# Autodesk Inventor assembly: ウィングユニット
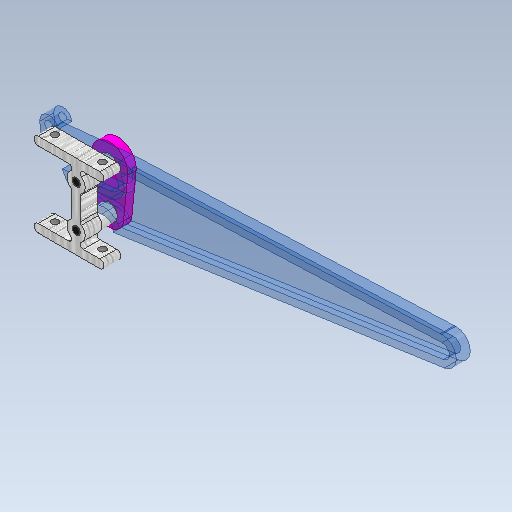
[picture p0: Inventor's stored thumbnail of the model, 512x512]
Saved by Autodesk Inventor 2020.2 (Build 242310000, 310)
## iProperties
Created: 2020-04-20
Part Number: ウィングユニット
Document SubType Name: Assembly
Designer: aoyama
Mass: 14.4308 g
Surface Area: 106.096 cm^2
Volume: 8.3252 cm^3
Density: 1.73339 g/cm^3
Author: aoyama
## Documents named in this file (6)
- C:\Users\aoyam\Desktop\SRDC_local\Inventor\二年機\Geminiβ\翼\WingUnitL.iam
- C:\Users\aoyam\Desktop\SRDC_local\Inventor\二年機\Geminiβ\翼\ウィング.ipt
- C:\Users\aoyam\Desktop\SRDC_local\Inventor\二年機\Geminiβ\翼\ウィング土台.ipt
- C:\Users\aoyam\Desktop\SRDC_local\Inventor\二年機\Geminiβ\翼\ウィング抑え.ipt
- C:\Users\aoyam\Desktop\SRDC_local\Inventor\二年機\Geminiβ\汎用部品\スペーサー中空M3L6アルミ.ipt
- C:\Users\aoyam\Desktop\SRDC_local\Inventor\二年機\Geminiβ\汎用部品\ネジボタンM3L15.ipt
## Components (7 placed, 5 different names)
1. ウィング:1 — 挿入:1
2. ウィング土台:1 — 挿入:1, 挿入:2, 挿入:3
3. ウィング抑え:1 — 挿入:4, 挿入:5, 挿入:6, 挿入:7
4. スペーサー中空M3L6アルミ:1 — 挿入:2, 挿入:4
5. スペーサー中空M3L6アルミ:2 — 挿入:3, 挿入:5
6. ネジボタンM3L15:1 — 挿入:6
7. ネジボタンM3L15:2 — 挿入:7
## Relationships (7: Insert 7)
- 挿入:1 [Insert]: ウィング:1 ↔ ウィング土台:1
- 挿入:2 [Insert]: ウィング土台:1 ↔ スペーサー中空M3L6アルミ:1
- 挿入:3 [Insert]: ウィング土台:1 ↔ スペーサー中空M3L6アルミ:2
- 挿入:4 [Insert]: ウィング抑え:1 ↔ スペーサー中空M3L6アルミ:1
- 挿入:5 [Insert]: ウィング抑え:1 ↔ スペーサー中空M3L6アルミ:2
- 挿入:6 [Insert]: ウィング抑え:1 ↔ ネジボタンM3L15:1
- 挿入:7 [Insert]: ウィング抑え:1 ↔ ネジボタンM3L15:2
